# Autodesk Inventor assembly: Z Axis Assembly
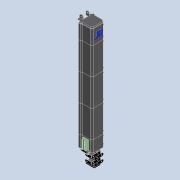
[picture p0: Inventor's stored thumbnail of the model, 180x180]
Saved by Autodesk Inventor 2022 (Build 260153000, 153)
## iProperties
Created: 2021-10-26
Part Number: Z Axis Assembly
Document SubType Name: Assembly
Designer: Coy
Author: Coy
## Documents named in this file (14)
- H:\3D Files\Project 3D Models\Breakfast Maker 2000\Assemblys\Z Axis Assembly.iam
- H:\3D Files\Project 3D Models\Breakfast Maker 2000\Linear Actuators\Z Axis Vertical Actuator.ipt
- H:\3D Files\Project 3D Models\Breakfast Maker 2000\3D Printed Parts\Z Axis Limt Adjustable Trigger.ipt
- H:\3D Files\Project 3D Models\Breakfast Maker 2000\3D Printed Parts\Z Axis Housing Frame Top Frunt.ipt
- H:\3D Files\Project 3D Models\Breakfast Maker 2000\Thread Inserts\M5 7mm OD 6mm Deep Threaded Insert.ipt
- H:\3D Files\Project 3D Models\Breakfast Maker 2000\Nuts and Bolts\M5 x 8 Pin Head Allen Bolt.ipt
- H:\3D Files\Project 3D Models\Breakfast Maker 2000\3D Printed Parts\Z Axis Cover Top Logo.ipt
- H:\3D Files\Project 3D Models\Breakfast Maker 2000\3D Printed Parts\Z Axis Cover Frame.ipt
- H:\3D Files\Project 3D Models\Breakfast Maker 2000\3D Printed Parts\Z Axis Cover.ipt
- H:\3D Files\Project 3D Models\Breakfast Maker 2000\3D Printed Parts\Z Axis Cover Frame Bottom.ipt
- H:\3D Files\Project 3D Models\Breakfast Maker 2000\3D Printed Parts\Z Axis Cover Bottom.ipt
- H:\3D Files\Project 3D Models\Breakfast Maker 2000\3D Printed Parts\JR Logo Text.ipt
- H:\3D Files\Project 3D Models\Breakfast Maker 2000\25Pin D SUB Female Connector.ipt
- H:\3D Files\Project 3D Models\Breakfast Maker 2000\90 deg Shelf 4 Hole Bracket.ipt
## Components (78 placed, 13 different names)
1. Z Axis Vertical Actuator:1 — Mate:1, Mate:2, Mate:3, Flush:2, Mate:22, Mate:25, Mate:28, Mate:80, Mate:81, Mate:82, Mate:83, Flush:44, Mate:90, Mate:111, Mate:112, Mate:113, Mate:114
2. Z Axis Limt Adjustable Trigger:1 — Mate:1, Mate:2, Flush:44
3. Z Axis Housing Frame Top Frunt:1 — Mate:3, Flush:2, Mate:5, Flush:3, Mate:6, Flush:4, Flush:5, Flush:6, Mate:9, Mate:10, Mate:11, Mate:12, Mate:13, Mate:14, Mate:15, Mate:16, Mate:17, Mate:18, Mate:24, Mate:80
4. M5 7mm OD 6mm Deep Threaded Insert:1 — Mate:5, Flush:3
5. M5 7mm OD 6mm Deep Threaded Insert:2 — Flush:6, Mate:18, Mate:21
6. M5 7mm OD 6mm Deep Threaded Insert:3 — Mate:6, Flush:4, Mate:20
7. M5 7mm OD 6mm Deep Threaded Insert:4 — Flush:5, Mate:17
8. M5 x 8 Pin Head Allen Bolt:1 — Mate:11, Mate:14
9. M5 x 8 Pin Head Allen Bolt:2 — Mate:9, Mate:16
10. M5 x 8 Pin Head Allen Bolt:3 — Mate:10, Mate:13
11. M5 x 8 Pin Head Allen Bolt:4 — Mate:12, Mate:15
12. Z Axis Cover Top Logo:1 — Mate:20, Mate:21, Mate:62, Mate:63, Mate:70, Mate:71, Mate:78, Mate:79, Mate:109
13. Z Axis Cover Frame:1 — Mate:22, Mate:24, Mate:27, Mate:31, Mate:33, Flush:7, Flush:8, Flush:9, Flush:10, Mate:43, Mate:44, Mate:45, Mate:46, Mate:55, Mate:81, Mate:85, Flush:45
14. Z Axis Cover Frame:2 — Mate:25, Mate:27, Mate:30, Mate:35, Mate:37, Flush:11, Flush:12, Flush:13, Flush:15, Mate:47, Mate:48, Mate:49, Mate:50, Mate:82, Mate:87, Flush:46
15. Z Axis Cover Frame:3 — Mate:28, Mate:30, Mate:39, Mate:41, Flush:14, Flush:16, Flush:17, Flush:18, Mate:51, Mate:52, Mate:53, Mate:54, Mate:83, Mate:89, Flush:47, Flush:48, Mate:91
16. Z Axis Cover:1 — Mate:56, Mate:57, Mate:64, Mate:65, Mate:72, Mate:73
17. Z Axis Cover:2 — Mate:58, Mate:59, Mate:66, Mate:67, Mate:74, Mate:75
18. Z Axis Cover:3 — Mate:60, Mate:61, Mate:68, Mate:69, Mate:76, Mate:77
19. M5 7mm OD 6mm Deep Threaded Insert:5 — Mate:31, Flush:7, Mate:56
20. M5 7mm OD 6mm Deep Threaded Insert:6 — Flush:10, Mate:57
21. M5 7mm OD 6mm Deep Threaded Insert:7 — Flush:8, Mate:84, Mate:85, Flush:45
22. M5 7mm OD 6mm Deep Threaded Insert:8 — Mate:33, Flush:9
23. M5 7mm OD 6mm Deep Threaded Insert:9 — Flush:12, Mate:86, Mate:87, Flush:46
24. M5 7mm OD 6mm Deep Threaded Insert:10 — Flush:15, Mate:59
25. M5 7mm OD 6mm Deep Threaded Insert:11 — Mate:35, Flush:11, Mate:58
26. M5 7mm OD 6mm Deep Threaded Insert:12 — Mate:37, Flush:13
27. M5 7mm OD 6mm Deep Threaded Insert:13 — Mate:41, Flush:17
28. M5 7mm OD 6mm Deep Threaded Insert:14 — Flush:18, Mate:61
29. M5 7mm OD 6mm Deep Threaded Insert:15 — Mate:39, Flush:14, Mate:60
30. M5 7mm OD 6mm Deep Threaded Insert:16 — Flush:16, Mate:88, Mate:89, Flush:47
31. M5 x 8 Pin Head Allen Bolt:5 — Mate:54, Flush:29
32. M5 x 8 Pin Head Allen Bolt:6 — Mate:43, Flush:21, Mate:55
33. M5 x 8 Pin Head Allen Bolt:7 — Mate:53, Flush:28
34. M5 x 8 Pin Head Allen Bolt:8 — Mate:44, Flush:20
35. M5 x 8 Pin Head Allen Bolt:9 — Mate:52, Flush:27, Flush:28
36. M5 x 8 Pin Head Allen Bolt:10 — Mate:45, Flush:19, Flush:20, Flush:21, Flush:23, Flush:24
37. M5 x 8 Pin Head Allen Bolt:11 — Mate:50, Flush:26
38. M5 x 8 Pin Head Allen Bolt:12 — Mate:46, Flush:19, Flush:22
39. M5 x 8 Pin Head Allen Bolt:13 — Mate:51, Flush:25, Flush:29
40. M5 x 8 Pin Head Allen Bolt:14 — Mate:47, Flush:23, Flush:25
41. M5 x 8 Pin Head Allen Bolt:15 — Mate:49, Flush:24, Flush:26, Flush:27
42. M5 x 8 Pin Head Allen Bolt:16 — Mate:48, Flush:22
43. M5 x 8 Pin Head Allen Bolt:17 — Mate:64, Flush:38, Flush:39
44. M5 x 8 Pin Head Allen Bolt:18 — Mate:65, Flush:39, Flush:40
45. M5 x 8 Pin Head Allen Bolt:19 — Mate:62, Flush:37, Mate:79
46. M5 x 8 Pin Head Allen Bolt:20 — Mate:63, Flush:37, Flush:38
47. M5 x 8 Pin Head Allen Bolt:21 — Mate:70, Flush:30, Flush:31, Mate:78
48. M5 x 8 Pin Head Allen Bolt:22 — Mate:77, Flush:36
49. M5 x 8 Pin Head Allen Bolt:23 — Mate:66, Flush:40, Flush:41
50. M5 x 8 Pin Head Allen Bolt:24 — Mate:67, Flush:41, Flush:42
51. M5 x 8 Pin Head Allen Bolt:25 — Mate:76, Flush:35, Flush:36, Mate:88
52. M5 x 8 Pin Head Allen Bolt:26 — Mate:75, Flush:34, Flush:35
53. M5 x 8 Pin Head Allen Bolt:27 — Mate:68, Flush:42, Flush:43
54. M5 x 8 Pin Head Allen Bolt:28 — Mate:69, Flush:43
55. M5 x 8 Pin Head Allen Bolt:29 — Mate:74, Flush:33, Flush:34, Mate:86
56. M5 x 8 Pin Head Allen Bolt:30 — Mate:73, Flush:32, Flush:33
57. M5 x 8 Pin Head Allen Bolt:31 — Mate:72, Flush:31, Flush:32, Mate:84
58. M5 x 8 Pin Head Allen Bolt:32 — Mate:71, Flush:30
59. Z Axis Cover Frame Bottom:1 — Mate:90, Flush:48, Mate:91, Mate:92, Mate:93, Mate:94, Mate:95, Mate:96, Mate:97, Mate:98, Mate:99, Flush:49, Flush:50, Flush:51, Flush:52, Mate:100
60. M5 7mm OD 6mm Deep Threaded Insert:17 — Mate:98, Flush:50
61. M5 7mm OD 6mm Deep Threaded Insert:18 — Mate:99, Flush:49, Mate:102
62. M5 7mm OD 6mm Deep Threaded Insert:19 — Mate:97, Flush:52
63. M5 7mm OD 6mm Deep Threaded Insert:20 — Mate:96, Flush:51, Mate:101
64. M5 x 8 Pin Head Allen Bolt:33 — Mate:92, Flush:53, Flush:54, Flush:55, Mate:100
65. M5 x 8 Pin Head Allen Bolt:34 — Mate:106, Flush:57
66. M5 x 8 Pin Head Allen Bolt:35 — Mate:104, Flush:56
67. M5 x 8 Pin Head Allen Bolt:36 — Mate:105, Flush:57, Mate:108
68. M5 x 8 Pin Head Allen Bolt:37 — Mate:95, Flush:53
69. M5 x 8 Pin Head Allen Bolt:38 — Mate:103, Flush:56, Mate:107
70. M5 x 8 Pin Head Allen Bolt:39 — Mate:93, Flush:54
71. M5 x 8 Pin Head Allen Bolt:40 — Mate:94, Flush:55
72. Z Axis Cover Bottom:1 — Mate:101, Mate:102, Mate:103, Mate:104, Mate:105, Mate:106, Mate:107, Mate:108, Mate:110, Flush:58
73. JR Logo Text:1 — Mate:109
74. 25Pin D SUB Female Connector:1 — Mate:110, Flush:58
75. 90 deg Shelf 4 Hole Bracket:1 — Mate:111, Flush:60
76. 90 deg Shelf 4 Hole Bracket:2 — Mate:112, Flush:60
77. 90 deg Shelf 4 Hole Bracket:3 — Mate:114, Flush:59
78. 90 deg Shelf 4 Hole Bracket:4 — Mate:113, Flush:59
## Relationships (160: Mate 101, Flush 59)
- Mate:1: Z Axis Vertical Actuator:1 ↔ Z Axis Limt Adjustable Trigger:1
- Mate:2 (102 mm): Z Axis Vertical Actuator:1 ↔ Z Axis Limt Adjustable Trigger:1
- Mate:3: Z Axis Vertical Actuator:1 ↔ Z Axis Housing Frame Top Frunt:1
- Flush:2 (-1 mm): Z Axis Vertical Actuator:1 ↔ Z Axis Housing Frame Top Frunt:1
- Mate:5: Z Axis Housing Frame Top Frunt:1 ↔ M5 7mm OD 6mm Deep Threaded Insert:1
- Flush:3: Z Axis Housing Frame Top Frunt:1 ↔ M5 7mm OD 6mm Deep Threaded Insert:1
- Mate:6: Z Axis Housing Frame Top Frunt:1 ↔ M5 7mm OD 6mm Deep Threaded Insert:3
- Flush:4: Z Axis Housing Frame Top Frunt:1 ↔ M5 7mm OD 6mm Deep Threaded Insert:3
- Flush:5: Z Axis Housing Frame Top Frunt:1 ↔ M5 7mm OD 6mm Deep Threaded Insert:4
- Flush:6: Z Axis Housing Frame Top Frunt:1 ↔ M5 7mm OD 6mm Deep Threaded Insert:2
- Mate:9: Z Axis Housing Frame Top Frunt:1 ↔ M5 x 8 Pin Head Allen Bolt:2
- Mate:10: Z Axis Housing Frame Top Frunt:1 ↔ M5 x 8 Pin Head Allen Bolt:3
- Mate:11: Z Axis Housing Frame Top Frunt:1 ↔ M5 x 8 Pin Head Allen Bolt:1
- Mate:12: Z Axis Housing Frame Top Frunt:1 ↔ M5 x 8 Pin Head Allen Bolt:4
- Mate:13: Z Axis Housing Frame Top Frunt:1 ↔ M5 x 8 Pin Head Allen Bolt:3
- Mate:14: Z Axis Housing Frame Top Frunt:1 ↔ M5 x 8 Pin Head Allen Bolt:1
- Mate:15: Z Axis Housing Frame Top Frunt:1 ↔ M5 x 8 Pin Head Allen Bolt:4
- Mate:16: Z Axis Housing Frame Top Frunt:1 ↔ M5 x 8 Pin Head Allen Bolt:2
- Mate:17: Z Axis Housing Frame Top Frunt:1 ↔ M5 7mm OD 6mm Deep Threaded Insert:4
- Mate:18: Z Axis Housing Frame Top Frunt:1 ↔ M5 7mm OD 6mm Deep Threaded Insert:2
- Mate:20: M5 7mm OD 6mm Deep Threaded Insert:3 ↔ Z Axis Cover Top Logo:1
- Mate:21: M5 7mm OD 6mm Deep Threaded Insert:2 ↔ Z Axis Cover Top Logo:1
- Mate:22: Z Axis Vertical Actuator:1 ↔ Z Axis Cover Frame:1
- Mate:24: Z Axis Housing Frame Top Frunt:1 ↔ Z Axis Cover Frame:1
- Mate:25: Z Axis Vertical Actuator:1 ↔ Z Axis Cover Frame:2
- Mate:27: Z Axis Cover Frame:1 ↔ Z Axis Cover Frame:2
- Mate:28: Z Axis Vertical Actuator:1 ↔ Z Axis Cover Frame:3
- Mate:30: Z Axis Cover Frame:2 ↔ Z Axis Cover Frame:3
- Mate:31: Z Axis Cover Frame:1 ↔ M5 7mm OD 6mm Deep Threaded Insert:5
- Mate:33: Z Axis Cover Frame:1 ↔ M5 7mm OD 6mm Deep Threaded Insert:8
- Mate:35: Z Axis Cover Frame:2 ↔ M5 7mm OD 6mm Deep Threaded Insert:11
- Mate:37: Z Axis Cover Frame:2 ↔ M5 7mm OD 6mm Deep Threaded Insert:12
- Mate:39: Z Axis Cover Frame:3 ↔ M5 7mm OD 6mm Deep Threaded Insert:15
- Mate:41: Z Axis Cover Frame:3 ↔ M5 7mm OD 6mm Deep Threaded Insert:13
- Flush:7: Z Axis Cover Frame:1 ↔ M5 7mm OD 6mm Deep Threaded Insert:5
- Flush:8: Z Axis Cover Frame:1 ↔ M5 7mm OD 6mm Deep Threaded Insert:7
- Flush:9: Z Axis Cover Frame:1 ↔ M5 7mm OD 6mm Deep Threaded Insert:8
- Flush:10: Z Axis Cover Frame:1 ↔ M5 7mm OD 6mm Deep Threaded Insert:6
- Flush:11: Z Axis Cover Frame:2 ↔ M5 7mm OD 6mm Deep Threaded Insert:11
- Flush:12: Z Axis Cover Frame:2 ↔ M5 7mm OD 6mm Deep Threaded Insert:9
- Flush:13: Z Axis Cover Frame:2 ↔ M5 7mm OD 6mm Deep Threaded Insert:12
- Flush:14: Z Axis Cover Frame:3 ↔ M5 7mm OD 6mm Deep Threaded Insert:15
- Flush:15: Z Axis Cover Frame:2 ↔ M5 7mm OD 6mm Deep Threaded Insert:10
- Flush:16: Z Axis Cover Frame:3 ↔ M5 7mm OD 6mm Deep Threaded Insert:16
- Flush:17: Z Axis Cover Frame:3 ↔ M5 7mm OD 6mm Deep Threaded Insert:13
- Flush:18: Z Axis Cover Frame:3 ↔ M5 7mm OD 6mm Deep Threaded Insert:14
- Mate:43: Z Axis Cover Frame:1 ↔ M5 x 8 Pin Head Allen Bolt:6
- Mate:44: Z Axis Cover Frame:1 ↔ M5 x 8 Pin Head Allen Bolt:8
- Mate:45: Z Axis Cover Frame:1 ↔ M5 x 8 Pin Head Allen Bolt:10
- Mate:46: Z Axis Cover Frame:1 ↔ M5 x 8 Pin Head Allen Bolt:12
- Mate:47: Z Axis Cover Frame:2 ↔ M5 x 8 Pin Head Allen Bolt:14
- Mate:48: Z Axis Cover Frame:2 ↔ M5 x 8 Pin Head Allen Bolt:16
- Mate:49: Z Axis Cover Frame:2 ↔ M5 x 8 Pin Head Allen Bolt:15
- Mate:50: Z Axis Cover Frame:2 ↔ M5 x 8 Pin Head Allen Bolt:11
- Mate:51: Z Axis Cover Frame:3 ↔ M5 x 8 Pin Head Allen Bolt:13
- Mate:52: Z Axis Cover Frame:3 ↔ M5 x 8 Pin Head Allen Bolt:9
- Mate:53: Z Axis Cover Frame:3 ↔ M5 x 8 Pin Head Allen Bolt:7
- Mate:54: Z Axis Cover Frame:3 ↔ M5 x 8 Pin Head Allen Bolt:5
- Flush:19: M5 x 8 Pin Head Allen Bolt:10 ↔ M5 x 8 Pin Head Allen Bolt:12
- Flush:20: M5 x 8 Pin Head Allen Bolt:8 ↔ M5 x 8 Pin Head Allen Bolt:10
- Flush:21: M5 x 8 Pin Head Allen Bolt:6 ↔ M5 x 8 Pin Head Allen Bolt:10
- Flush:22: M5 x 8 Pin Head Allen Bolt:12 ↔ M5 x 8 Pin Head Allen Bolt:16
- Flush:23: M5 x 8 Pin Head Allen Bolt:10 ↔ M5 x 8 Pin Head Allen Bolt:14
- Flush:24: M5 x 8 Pin Head Allen Bolt:10 ↔ M5 x 8 Pin Head Allen Bolt:15
- Flush:25: M5 x 8 Pin Head Allen Bolt:13 ↔ M5 x 8 Pin Head Allen Bolt:14
- Flush:26: M5 x 8 Pin Head Allen Bolt:11 ↔ M5 x 8 Pin Head Allen Bolt:15
- Flush:27: M5 x 8 Pin Head Allen Bolt:9 ↔ M5 x 8 Pin Head Allen Bolt:15
- Flush:28: M5 x 8 Pin Head Allen Bolt:7 ↔ M5 x 8 Pin Head Allen Bolt:9
- Flush:29: M5 x 8 Pin Head Allen Bolt:5 ↔ M5 x 8 Pin Head Allen Bolt:13
- Mate:55: Z Axis Cover Frame:1 ↔ M5 x 8 Pin Head Allen Bolt:6
- Mate:56: Z Axis Cover:1 ↔ M5 7mm OD 6mm Deep Threaded Insert:5
- Mate:57: Z Axis Cover:1 ↔ M5 7mm OD 6mm Deep Threaded Insert:6
- Mate:58: Z Axis Cover:2 ↔ M5 7mm OD 6mm Deep Threaded Insert:11
- Mate:59: Z Axis Cover:2 ↔ M5 7mm OD 6mm Deep Threaded Insert:10
- Mate:60: Z Axis Cover:3 ↔ M5 7mm OD 6mm Deep Threaded Insert:15
- Mate:61: Z Axis Cover:3 ↔ M5 7mm OD 6mm Deep Threaded Insert:14
- Mate:62: Z Axis Cover Top Logo:1 ↔ M5 x 8 Pin Head Allen Bolt:19
- Mate:63: Z Axis Cover Top Logo:1 ↔ M5 x 8 Pin Head Allen Bolt:20
- Mate:64: Z Axis Cover:1 ↔ M5 x 8 Pin Head Allen Bolt:17
- Mate:65: Z Axis Cover:1 ↔ M5 x 8 Pin Head Allen Bolt:18
- Mate:66: Z Axis Cover:2 ↔ M5 x 8 Pin Head Allen Bolt:23
- Mate:67: Z Axis Cover:2 ↔ M5 x 8 Pin Head Allen Bolt:24
- Mate:68: Z Axis Cover:3 ↔ M5 x 8 Pin Head Allen Bolt:27
- Mate:69: Z Axis Cover:3 ↔ M5 x 8 Pin Head Allen Bolt:28
- Mate:70: Z Axis Cover Top Logo:1 ↔ M5 x 8 Pin Head Allen Bolt:21
- Mate:71: Z Axis Cover Top Logo:1 ↔ M5 x 8 Pin Head Allen Bolt:32
- Mate:72: Z Axis Cover:1 ↔ M5 x 8 Pin Head Allen Bolt:31
- Mate:73: Z Axis Cover:1 ↔ M5 x 8 Pin Head Allen Bolt:30
- Mate:74: Z Axis Cover:2 ↔ M5 x 8 Pin Head Allen Bolt:29
- Mate:75: Z Axis Cover:2 ↔ M5 x 8 Pin Head Allen Bolt:26
- Mate:76: Z Axis Cover:3 ↔ M5 x 8 Pin Head Allen Bolt:25
- Mate:77: Z Axis Cover:3 ↔ M5 x 8 Pin Head Allen Bolt:22
- Flush:30: M5 x 8 Pin Head Allen Bolt:21 ↔ M5 x 8 Pin Head Allen Bolt:32
- Flush:31: M5 x 8 Pin Head Allen Bolt:21 ↔ M5 x 8 Pin Head Allen Bolt:31
- Flush:32: M5 x 8 Pin Head Allen Bolt:30 ↔ M5 x 8 Pin Head Allen Bolt:31
- Flush:33: M5 x 8 Pin Head Allen Bolt:29 ↔ M5 x 8 Pin Head Allen Bolt:30
- Flush:34: M5 x 8 Pin Head Allen Bolt:26 ↔ M5 x 8 Pin Head Allen Bolt:29
- Flush:35: M5 x 8 Pin Head Allen Bolt:25 ↔ M5 x 8 Pin Head Allen Bolt:26
- Flush:36: M5 x 8 Pin Head Allen Bolt:22 ↔ M5 x 8 Pin Head Allen Bolt:25
- Mate:78: Z Axis Cover Top Logo:1 ↔ M5 x 8 Pin Head Allen Bolt:21
- Flush:37: M5 x 8 Pin Head Allen Bolt:19 ↔ M5 x 8 Pin Head Allen Bolt:20
- Flush:38: M5 x 8 Pin Head Allen Bolt:17 ↔ M5 x 8 Pin Head Allen Bolt:20
- Flush:39: M5 x 8 Pin Head Allen Bolt:17 ↔ M5 x 8 Pin Head Allen Bolt:18
- Flush:40: M5 x 8 Pin Head Allen Bolt:18 ↔ M5 x 8 Pin Head Allen Bolt:23
- Flush:41: M5 x 8 Pin Head Allen Bolt:23 ↔ M5 x 8 Pin Head Allen Bolt:24
- Flush:42: M5 x 8 Pin Head Allen Bolt:24 ↔ M5 x 8 Pin Head Allen Bolt:27
- Flush:43: M5 x 8 Pin Head Allen Bolt:27 ↔ M5 x 8 Pin Head Allen Bolt:28
- Mate:79: Z Axis Cover Top Logo:1 ↔ M5 x 8 Pin Head Allen Bolt:19
- Mate:80 (0.5 mm): Z Axis Vertical Actuator:1 ↔ Z Axis Housing Frame Top Frunt:1
- Mate:81 (9 mm): Z Axis Vertical Actuator:1 ↔ Z Axis Cover Frame:1
- Mate:82 (9 mm): Z Axis Vertical Actuator:1 ↔ Z Axis Cover Frame:2
- Mate:83 (9 mm): Z Axis Vertical Actuator:1 ↔ Z Axis Cover Frame:3
- Flush:44: Z Axis Vertical Actuator:1 ↔ Z Axis Limt Adjustable Trigger:1
- Mate:84: M5 7mm OD 6mm Deep Threaded Insert:7 ↔ M5 x 8 Pin Head Allen Bolt:31
- Mate:85: Z Axis Cover Frame:1 ↔ M5 7mm OD 6mm Deep Threaded Insert:7
- Flush:45: Z Axis Cover Frame:1 ↔ M5 7mm OD 6mm Deep Threaded Insert:7
- Mate:86: M5 7mm OD 6mm Deep Threaded Insert:9 ↔ M5 x 8 Pin Head Allen Bolt:29
- Mate:87: Z Axis Cover Frame:2 ↔ M5 7mm OD 6mm Deep Threaded Insert:9
- Flush:46: Z Axis Cover Frame:2 ↔ M5 7mm OD 6mm Deep Threaded Insert:9
- Mate:88: M5 7mm OD 6mm Deep Threaded Insert:16 ↔ M5 x 8 Pin Head Allen Bolt:25
- Mate:89: Z Axis Cover Frame:3 ↔ M5 7mm OD 6mm Deep Threaded Insert:16
- Flush:47: Z Axis Cover Frame:3 ↔ M5 7mm OD 6mm Deep Threaded Insert:16
- Mate:90: Z Axis Vertical Actuator:1 ↔ Z Axis Cover Frame Bottom:1
- Flush:48: Z Axis Cover Frame:3 ↔ Z Axis Cover Frame Bottom:1
- Mate:91: Z Axis Cover Frame:3 ↔ Z Axis Cover Frame Bottom:1
- Mate:92: Z Axis Cover Frame Bottom:1 ↔ M5 x 8 Pin Head Allen Bolt:33
- Mate:93: Z Axis Cover Frame Bottom:1 ↔ M5 x 8 Pin Head Allen Bolt:39
- Mate:94: Z Axis Cover Frame Bottom:1 ↔ M5 x 8 Pin Head Allen Bolt:40
- Mate:95: Z Axis Cover Frame Bottom:1 ↔ M5 x 8 Pin Head Allen Bolt:37
- Mate:96: Z Axis Cover Frame Bottom:1 ↔ M5 7mm OD 6mm Deep Threaded Insert:20
- Mate:97: Z Axis Cover Frame Bottom:1 ↔ M5 7mm OD 6mm Deep Threaded Insert:19
- Mate:98: Z Axis Cover Frame Bottom:1 ↔ M5 7mm OD 6mm Deep Threaded Insert:17
- Mate:99: Z Axis Cover Frame Bottom:1 ↔ M5 7mm OD 6mm Deep Threaded Insert:18
- Flush:49: Z Axis Cover Frame Bottom:1 ↔ M5 7mm OD 6mm Deep Threaded Insert:18
- Flush:50: Z Axis Cover Frame Bottom:1 ↔ M5 7mm OD 6mm Deep Threaded Insert:17
- Flush:51: Z Axis Cover Frame Bottom:1 ↔ M5 7mm OD 6mm Deep Threaded Insert:20
- Flush:52: Z Axis Cover Frame Bottom:1 ↔ M5 7mm OD 6mm Deep Threaded Insert:19
- Flush:53: M5 x 8 Pin Head Allen Bolt:33 ↔ M5 x 8 Pin Head Allen Bolt:37
- Flush:54: M5 x 8 Pin Head Allen Bolt:33 ↔ M5 x 8 Pin Head Allen Bolt:39
- Flush:55: M5 x 8 Pin Head Allen Bolt:33 ↔ M5 x 8 Pin Head Allen Bolt:40
- Mate:100: Z Axis Cover Frame Bottom:1 ↔ M5 x 8 Pin Head Allen Bolt:33
- Mate:101: M5 7mm OD 6mm Deep Threaded Insert:20 ↔ Z Axis Cover Bottom:1
- Mate:102: M5 7mm OD 6mm Deep Threaded Insert:18 ↔ Z Axis Cover Bottom:1
- Mate:103: M5 x 8 Pin Head Allen Bolt:38 ↔ Z Axis Cover Bottom:1
- Mate:104: M5 x 8 Pin Head Allen Bolt:35 ↔ Z Axis Cover Bottom:1
- Mate:105: M5 x 8 Pin Head Allen Bolt:36 ↔ Z Axis Cover Bottom:1
- Mate:106: M5 x 8 Pin Head Allen Bolt:34 ↔ Z Axis Cover Bottom:1
- Flush:56: M5 x 8 Pin Head Allen Bolt:35 ↔ M5 x 8 Pin Head Allen Bolt:38
- Mate:107: M5 x 8 Pin Head Allen Bolt:38 ↔ Z Axis Cover Bottom:1
- Flush:57: M5 x 8 Pin Head Allen Bolt:34 ↔ M5 x 8 Pin Head Allen Bolt:36
- Mate:108: M5 x 8 Pin Head Allen Bolt:36 ↔ Z Axis Cover Bottom:1
- Mate:109: Z Axis Cover Top Logo:1 ↔ JR Logo Text:1
- Mate:110: Z Axis Cover Bottom:1 ↔ 25Pin D SUB Female Connector:1
- Flush:58 (-3 mm): Z Axis Cover Bottom:1 ↔ 25Pin D SUB Female Connector:1
- Mate:111: Z Axis Vertical Actuator:1 ↔ 90 deg Shelf 4 Hole Bracket:1
- Mate:112: Z Axis Vertical Actuator:1 ↔ 90 deg Shelf 4 Hole Bracket:2
- Mate:113: Z Axis Vertical Actuator:1 ↔ 90 deg Shelf 4 Hole Bracket:4
- Mate:114: Z Axis Vertical Actuator:1 ↔ 90 deg Shelf 4 Hole Bracket:3
- Flush:59: 90 deg Shelf 4 Hole Bracket:3 ↔ 90 deg Shelf 4 Hole Bracket:4
- Flush:60: 90 deg Shelf 4 Hole Bracket:1 ↔ 90 deg Shelf 4 Hole Bracket:2
